# Autodesk Inventor assembly: right-side-front-mechanism_MIR
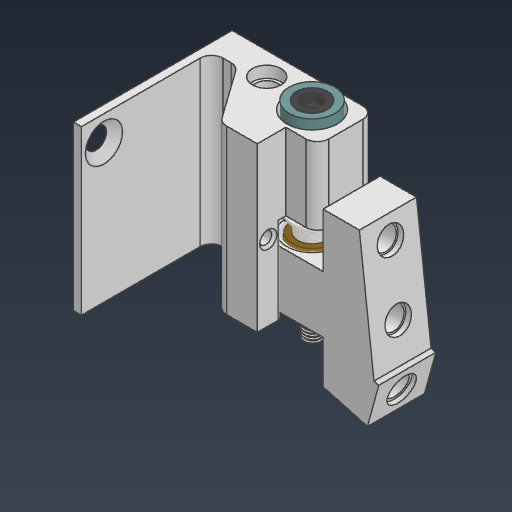
[picture p0: Inventor's stored thumbnail of the model, 512x512]
Saved by Autodesk Inventor 2023 (Build 270158000, 158)
## iProperties
Created: 2025-04-06
Part Number: right-side-front-mechanism_MIR
Document SubType Name: Assembly
Designer: szymo
Mass: 14.0827 g
Surface Area: 83.2214 cm^2
Volume: 8.99579 cm^3
Density: 1.56548 g/cm^3
Author: szymo
## Documents named in this file (4)
- D:\tech\robotyka\robots\evangelion\inventor-project\right-side-front-mechanism_MIR.iam
- D:\tech\robotyka\robots\evangelion\inventor-project\front-mechanizm_MIR.iam
- D:\tech\robotyka\robots\evangelion\inventor-project\side-right_MIR.ipt
- D:\tech\robotyka\robots\evangelion\inventor-project\front-fight-holder_MIR.ipt
## Components (3 placed, 3 different names)
1. front-mechanizm_MIR:1 [sub-assembly] — Tangent:1
2. side-right_MIR:1
3. front-fight-holder_MIR:1 — Tangent:1
## Relationships (1: Tangent 1)
- Tangent:1 (2.5 mm): front-mechanizm_MIR:1 ↔ front-fight-holder_MIR:1
